# Autodesk Inventor assembly: engranajes motor hombro dimer 3.1
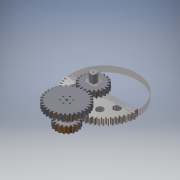
[picture p0: Inventor's stored thumbnail of the model, 180x180]
Saved by Autodesk Inventor 2016 (Build 200138000, 138)
## iProperties
Created: 2016-06-23
Part Number: engranajes motor hombro dimer 3.1
Document SubType Name: Assembly
Designer: Admin
Author: Admin
## Documents named in this file (9)
- C:\Users\Admin\Documents\diseños autodesk dimer\engranajes dimer hombro muelles\engranajes motor hombro dimer 3.1.iam
- C:\Users\Admin\Desktop\engranajes motor hombro dimer 3.1\Design Accelerator\Spur Gears1.iam
- C:\Users\Admin\Desktop\engranajes motor hombro dimer 3.1\Design Accelerator\Spur Gears3.iam
- C:\Users\Admin\Documents\diseños autodesk dimer\engranajes dimer hombro muelles\perfil aluminio.ipt
- C:\Users\Admin\Documents\diseños autodesk dimer\engranajes dimer hombro muelles\caja perfil.ipt
- C:\Users\Admin\Documents\diseños autodesk dimer\engranajes dimer hombro muelles\eje motor.ipt
- C:\Users\Admin\Documents\diseños autodesk dimer\engranajes dimer hombro muelles\engranajes motor hombro dimer 3.1\Design Accelerator\Spur Gears1.iam
- C:\Users\Admin\Documents\diseños autodesk dimer\engranajes dimer hombro muelles\engranajes motor hombro dimer 3.1\Design Accelerator\Spur Gears2.iam
- C:\Users\Admin\Documents\diseños autodesk dimer\engranajes dimer hombro muelles\eje union engrane reductor.ipt
## Components (8 placed, 8 different names)
1. piñon motor [sub-assembly] — Flush:7, Mate:4, Tangent:1, Rotation:1, Mate:9
2. engrane brazo [sub-assembly] — Mate:2, Flush:3, Tangent:2, Flush:9
3. perfil aluminio:1 — Flush:4, Flush:5, Flush:6
4. caja perfil:1 — Mate:2, Flush:3, Flush:4, Flush:5, Flush:6
5. eje motor:1 — Flush:7, Mate:4
6. reductor motor [sub-assembly] — Mate:5, Mate:6, Mate:7, Tangent:1, Rotation:1, Mate:9
7. reductor brazo [sub-assembly] — Mate:5, Mate:6, Mate:8, Tangent:2, Flush:9
8. eje union engrane reductor:1 — Mate:7, Mate:8
## Relationships (16: Mate 7, Flush 6, Tangent 2, RelateRotation 1)
- Mate:2 (-8.5 mm): engrane brazo ↔ caja perfil:1
- Flush:3: engrane brazo ↔ caja perfil:1
- Flush:4 (2.5 mm): perfil aluminio:1 ↔ caja perfil:1
- Flush:5 (2.5 mm): perfil aluminio:1 ↔ caja perfil:1
- Flush:6 (-100 mm): perfil aluminio:1 ↔ caja perfil:1
- Flush:7: piñon motor ↔ eje motor:1
- Mate:4: piñon motor ↔ eje motor:1
- Mate:5: reductor motor ↔ reductor brazo
- Mate:6 (26 mm): reductor motor ↔ reductor brazo
- Mate:7: reductor motor ↔ eje union engrane reductor:1
- Tangent:1: piñon motor ↔ reductor motor
- Rotation:1 [RelateRotation] (1 ul): piñon motor ↔ reductor motor
- Mate:8: reductor brazo ↔ eje union engrane reductor:1
- Tangent:2: engrane brazo ↔ reductor brazo
- Flush:9: engrane brazo ↔ reductor brazo
- Mate:9 (-15 mm): piñon motor ↔ reductor motor
